# Autodesk Inventor assembly: Arduino MEGA2650
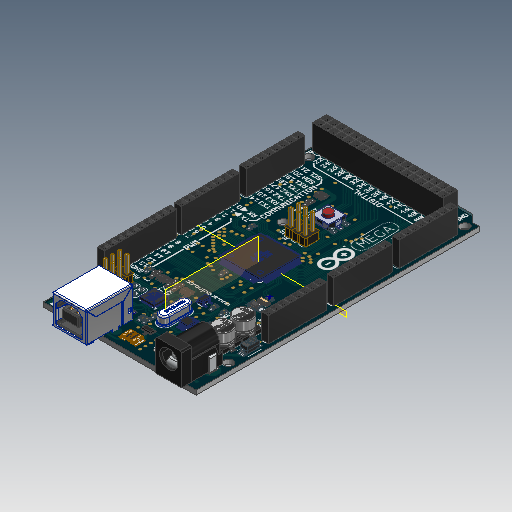
[picture p0: Inventor's stored thumbnail of the model, 512x512]
Saved by Autodesk Inventor 2017 (Build 210142000, 142)
## iProperties
Created: 2013-12-29
Part Number: Arduino MEGA2650
Document SubType Name: Ensemble
Mass: 33.6534 g
Surface Area: 264.487 cm^2
Volume: 16.1511 cm^3
Density: 2.08366 g/cm^3
Stock Number: 1420-11-10
Sending System: SolidWorks 2012
Last Author: A
Last Saved: 2014-01-03
## Documents named in this file (30)
- W:\Professionnel\Conception FABLAB\1420-Vauban 3D XL\1420-11 Electronique\1420-11-10 Arduino\1420-11-10 Arduino Mega.iam
- W:\Professionnel\Conception FABLAB\1420-Vauban 3D XL\1420-11 Electronique\1420-11-10 Arduino\MEGAboard.ipt
- W:\Professionnel\Conception FABLAB\1420-Vauban 3D XL\1420-11 Electronique\1420-11-10 Arduino\47uf CAP Dcase.ipt
- W:\Professionnel\Conception FABLAB\1420-Vauban 3D XL\1420-11 Electronique\1420-11-10 Arduino\USB type b.SLDPRT.iam
- W:\Professionnel\Conception FABLAB\1420-Vauban 3D XL\1420-11 Electronique\1420-11-10 Arduino\power jack.ipt
- W:\Professionnel\Conception FABLAB\1420-Vauban 3D XL\1420-11 Electronique\1420-11-10 Arduino\crystal.ipt
- W:\Professionnel\Conception FABLAB\1420-Vauban 3D XL\1420-11 Electronique\1420-11-10 Arduino\2pin_header__02.ipt
- W:\Professionnel\Conception FABLAB\1420-Vauban 3D XL\1420-11 Electronique\1420-11-10 Arduino\reg.ipt
- W:\Professionnel\Conception FABLAB\1420-Vauban 3D XL\1420-11 Electronique\1420-11-10 Arduino\led.ipt
- W:\Professionnel\Conception FABLAB\1420-Vauban 3D XL\1420-11 Electronique\1420-11-10 Arduino\atmega16u2.ipt
- W:\Professionnel\Conception FABLAB\1420-Vauban 3D XL\1420-11 Electronique\1420-11-10 Arduino\8 PORT HEADER.ipt
- W:\Professionnel\Conception FABLAB\1420-Vauban 3D XL\1420-11 Electronique\1420-11-10 Arduino\10 PORT HEADER.ipt
- W:\Professionnel\Conception FABLAB\1420-Vauban 3D XL\1420-11 Electronique\1420-11-10 Arduino\102 RESISTOR PACK.ipt
- W:\Professionnel\Conception FABLAB\1420-Vauban 3D XL\1420-11 Electronique\1420-11-10 Arduino\103 RESISTOR PACK.ipt
- W:\Professionnel\Conception FABLAB\1420-Vauban 3D XL\1420-11 Electronique\1420-11-10 Arduino\220 RESISTOR PACK.ipt
- W:\Professionnel\Conception FABLAB\1420-Vauban 3D XL\1420-11 Electronique\1420-11-10 Arduino\16mhz crystal - measured.ipt
- W:\Professionnel\Conception FABLAB\1420-Vauban 3D XL\1420-11 Electronique\1420-11-10 Arduino\PADS001.ipt
- W:\Professionnel\Conception FABLAB\1420-Vauban 3D XL\1420-11 Electronique\1420-11-10 Arduino\603 cap on pad.ipt
- W:\Professionnel\Conception FABLAB\1420-Vauban 3D XL\1420-11 Electronique\1420-11-10 Arduino\ssot3.ipt
- W:\Professionnel\Conception FABLAB\1420-Vauban 3D XL\1420-11 Electronique\1420-11-10 Arduino\mf-msmf050-2.ipt
- W:\Professionnel\Conception FABLAB\1420-Vauban 3D XL\1420-11 Electronique\1420-11-10 Arduino\lmv358.ipt
- W:\Professionnel\Conception FABLAB\1420-Vauban 3D XL\1420-11 Electronique\1420-11-10 Arduino\lp2985dgkr.ipt
- W:\Professionnel\Conception FABLAB\1420-Vauban 3D XL\1420-11 Electronique\1420-11-10 Arduino\cd1206 diode.ipt
- W:\Professionnel\Conception FABLAB\1420-Vauban 3D XL\1420-11 Electronique\1420-11-10 Arduino\603 resistor.ipt
- W:\Professionnel\Conception FABLAB\1420-Vauban 3D XL\1420-11 Electronique\1420-11-10 Arduino\blm21.ipt
- W:\Professionnel\Conception FABLAB\1420-Vauban 3D XL\1420-11 Electronique\1420-11-10 Arduino\m7 diode.ipt
- W:\Professionnel\Conception FABLAB\1420-Vauban 3D XL\1420-11 Electronique\1420-11-10 Arduino\MLC0603.ipt
- W:\Professionnel\Conception FABLAB\1420-Vauban 3D XL\1420-11 Electronique\1420-11-10 Arduino\RESET BUTTON.iam
- W:\Professionnel\Conception FABLAB\1420-Vauban 3D XL\1420-11 Electronique\1420-11-10 Arduino\18 X 2 ROW HEADER.ipt
- W:\Professionnel\Conception FABLAB\1420-Vauban 3D XL\1420-11 Electronique\1420-11-10 Arduino\atmega2650-16AU.ipt
## Components (61 placed, 29 different names)
1. MEGAboard:1 — Affleurement:1
2. 47uf CAP Dcase:1
3. USB type b.SLDPRT:1 [sub-assembly]
4. power jack:1
5. 47uf CAP Dcase:2
6. crystal:1
7. 2pin_header__02:1
8. reg:1
9. led:1
10. 2pin_header__02:2
11. 2pin_header__02:3
12. 2pin_header__02:4
13. 2pin_header__02:5
14. 2pin_header__02:6
15. atmega16u2:1
16. led:2
17. led:3
18. led:4
19. 8 PORT HEADER:3
20. 8 PORT HEADER:4 — Symétrie:1
21. 8 PORT HEADER:6
22. 10 PORT HEADER:1 — Symétrie:1
23. 102 RESISTOR PACK:1
24. 102 RESISTOR PACK:2
25. 103 RESISTOR PACK:3
26. 220 RESISTOR PACK:1
27. 16mhz crystal - measured:1
28. PADS001:1
29. 603 cap on pad:1
30. ssot3:1
31. mf-msmf050-2:1
32. 603 cap on pad:2
33. 603 cap on pad:3
34. lmv358:1
35. 603 cap on pad:4
36. 603 cap on pad:5
37. 603 cap on pad:6
38. 603 cap on pad:7
39. 603 cap on pad:8
40. lp2985dgkr:1
41. cd1206 diode:1
42. cd1206 diode:2
43. 603 resistor:1
44. blm21:1
45. m7 diode:1
46. MLC0603:1
47. MLC0603:2
48. RESET BUTTON:1 [sub-assembly]
49. 8 PORT HEADER:5
50. 8 PORT HEADER:7
51. 603 cap on pad:9
52. 603 cap on pad:10
53. 103 RESISTOR PACK:4
54. 603 cap on pad:11
55. 603 cap on pad:12
56. 603 cap on pad:13
57. 603 resistor:2
58. 603 cap on pad:14
59. 603 cap on pad:15
60. 18 X 2 ROW HEADER:1
61. atmega2650-16AU:1
## Relationships (2: Symmetry 1, Flush 1)
- Symétrie:1 [Symmetry]: 8 PORT HEADER:4 ↔ 10 PORT HEADER:1
- Affleurement:1 [Flush] (-50 mm): MEGAboard:1
